# Autodesk Inventor assembly: Alliance Short Mogo
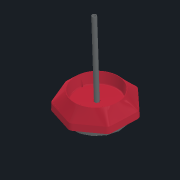
[picture p0: Inventor's stored thumbnail of the model, 180x180]
Saved by Autodesk Inventor 2021 (Build 250183000, 183)
## iProperties
Created: 2021-05-29
Part Number: Alliance Short Mogo
Document SubType Name: Assembly
Designer: max
Sending System: Autodesk Inventor 2021
Preprocessor: ST-DEVELOPER v18.1
Title: C:\Users\max\Desktop\Vex\TiP FieldCAD\Mogos\Alliance Short Mogo.stp
Author: max
Revision Number: ANY
## Documents named in this file (8)
- C:\Users\max\Desktop\Vex\TiP FieldCAD\Mogos\Red Alliance Mogo.iam
- C:\Users\max\Desktop\Vex\TiP FieldCAD\Mogos\Nut Nylock.ipt
- C:\Users\max\Desktop\Vex\TiP FieldCAD\Mogos\Mogo Post.ipt
- C:\Users\max\Desktop\Vex\TiP FieldCAD\Mogos\Mogo Base Post Grip.ipt
- C:\Users\max\Desktop\Vex\TiP FieldCAD\Mogos\Screw 8-32 Steel .625.ipt
- C:\Users\max\Desktop\Vex\TiP FieldCAD\Mogos\Mogo Base Bottom.ipt
- C:\Users\max\Desktop\Vex\TiP FieldCAD\Mogos\Mogo Base Weight.ipt
- C:\Users\max\Desktop\Vex\TiP FieldCAD\Mogos\Mogo Base Red.ipt
## Components (13 placed, 7 different names)
1. Mogo Post:1 — Mate:2, Mate:4
2. Mogo Base Post Grip:1
3. Mogo Base Post Grip:2
4. Nut Nylock:7
5. Screw 8-32 Steel .625:7
6. Nut Nylock:8
7. Screw 8-32 Steel .625:8
8. Nut Nylock:9
9. Nut Nylock:10
10. Nut Nylock:11 — Mate:5, Mate:6
11. Mogo Base Bottom:1 — Mate:1, Mate:3
12. Mogo Base Weight:1 — Mate:1, Mate:2, Mate:3
13. Mogo Base Red:1 — Mate:4, Mate:5, Mate:6
## Relationships (6: Mate 6)
- Mate:1: Mogo Base Bottom:1 ↔ Mogo Base Weight:1
- Mate:2: Mogo Post:1 ↔ Mogo Base Weight:1
- Mate:3: Mogo Base Bottom:1 ↔ Mogo Base Weight:1
- Mate:4: Mogo Post:1 ↔ Mogo Base Red:1
- Mate:5: Nut Nylock:11 ↔ Mogo Base Red:1
- Mate:6: Nut Nylock:11 ↔ Mogo Base Red:1
